# Autodesk Inventor assembly: replace
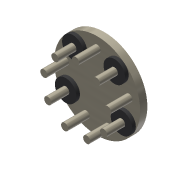
[picture p0: Inventor's stored thumbnail of the model, 180x180]
Saved by Autodesk Inventor 2022 Beta2 (Build 260130000, 130) ContinuousBuild 0
## iProperties
Shininess: 64.0
Length Units: 11272
Angle Units: 11279
Time Units: 11290
Mass Units: 11286
Length Display Precision: 3
Angle Display Precision: 2
Compacted: True
Part Number: replace
Document SubType Name: Assembly
Created: 2002-10-31
Designer: gbarnes
Density: 0.0
Volumn: 0.0
Area: 0.0
PropertySet Name: Model Information
Control State: 0
Master: False
Checked Out: False
Author: gbarnes
## Documents named in this file (3)
- C:\Autodesk Inventor 2021 Intro Practice Files\replace.iam
- C:\Autodesk Inventor 2021 Intro Practice Files\compholder.ipt
- C:\Autodesk Inventor 2021 Intro Practice Files\round.ipt
## Components (5 placed, 2 different names)
1. compholder:1 — Insert:1, Insert:2, Insert:3, Insert:4
2. round:1 — Insert:1
3. round:2 — Insert:2
4. round:3 — Insert:3
5. round:4 — Insert:4
## Relationships (4: Insert 4)
- Insert:1: compholder:1 ↔ round:1
- Insert:2: compholder:1 ↔ round:2
- Insert:3: compholder:1 ↔ round:3
- Insert:4: compholder:1 ↔ round:4
